# Autodesk Inventor assembly: Synchronous Belts Transmission
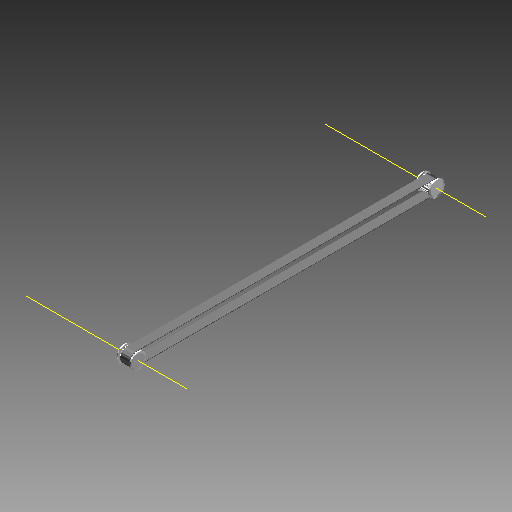
[picture p0: Inventor's stored thumbnail of the model, 512x512]
Saved by Autodesk Inventor 2019.4 (Build 234330000, 330)
## iProperties
Created: 2020-01-24
Part Number: Synchronous Belts Transmission
Document SubType Name: Assembly
Designer: admin
Mass: 178.465 g
Surface Area: 473.753 cm^2
Volume: 39.025 cm^3
Density: 4.57309 g/cm^3
ClientObjectVersion: 1
Author: admin
## Documents named in this file (4)
- C:\Users\Mark\Desktop\7738 Helion Engineering\7738-2020\Robot V2\Storage System\Storage System Assembly\Design Accelerator\Synchronous Belts Transmission6.iam
- C:\Users\Mark\Desktop\7738 Helion Engineering\7738-2020\Robot V2\Storage System\Storage System Assembly\Design Accelerator\Synchronous Belt6.ipt
- C:\Users\Mark\Desktop\7738 Helion Engineering\7738-2020\Robot V2\Storage System\Storage System Assembly\Design Accelerator\Synchronous Pulley16.ipt
- C:\Users\Mark\Desktop\7738 Helion Engineering\7738-2020\Robot V2\Storage System\Storage System Assembly\Design Accelerator\Synchronous Pulley26.ipt
## Components (3 placed, 3 different names)
1. Synchronous Belt:1 — Flush:1, Mate:1, Mate:2, Flush:2, Mate:3, Mate:4
2. Synchronous Pulley1:1 — Flush:1, Mate:1, Mate:2, Rotation:1
3. Synchronous Pulley2:1 — Flush:2, Mate:3, Rotation:1, Mate:4
## Relationships (7: Mate 4, Flush 2, RelateRotation 1)
- Flush:1: Synchronous Belt:1 ↔ Synchronous Pulley1:1
- Mate:1: Synchronous Belt:1 ↔ Synchronous Pulley1:1
- Mate:2: Synchronous Belt:1 ↔ Synchronous Pulley1:1
- Flush:2: Synchronous Belt:1 ↔ Synchronous Pulley2:1
- Mate:3: Synchronous Belt:1 ↔ Synchronous Pulley2:1
- Rotation:1 [RelateRotation] (1 ul): Synchronous Pulley1:1 ↔ Synchronous Pulley2:1
- Mate:4: Synchronous Belt:1 ↔ Synchronous Pulley2:1
